# Autodesk Inventor assembly: Motor + Shaft_MIR
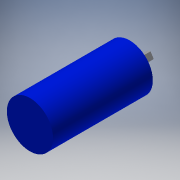
[picture p0: Inventor's stored thumbnail of the model, 180x180]
Saved by Autodesk Inventor 2016 SP1 (Build 200210100, 210)
## iProperties
Created: 2016-04-13
Part Number: Motor + Shaft_MIR
Document SubType Name: Assembly
Designer: schiu30
Author: schiu30
## Documents named in this file (3)
- \\prism.nas.gatech.edu\schiu30\vlab\desktop\Capstone\Capstone CAD\Capstone CAD\Motor + Attachment\Motor + Shaft_MIR.iam
- \\prism.nas.gatech.edu\schiu30\vlab\desktop\Capstone\Capstone CAD\Capstone CAD\Motor + Attachment\Motor Shaft_MIR.ipt
- \\prism.nas.gatech.edu\schiu30\vlab\desktop\Capstone\Capstone CAD\Capstone CAD\Motor + Attachment\Motor_MIR.ipt
## Components (2 placed, 2 different names)
1. Motor Shaft_MIR:1 — Insert:1
2. Motor_MIR:1 — Flush:3, Flush:2, Flush:1, Insert:1
## Relationships (4: Flush 3, Insert 1)
- Flush:3: Motor_MIR:1
- Flush:2: Motor_MIR:1
- Flush:1: Motor_MIR:1
- Insert:1: Motor Shaft_MIR:1 ↔ Motor_MIR:1
